# Autodesk Inventor assembly: Durometer_Vertical_Lead_Screw_Assembly
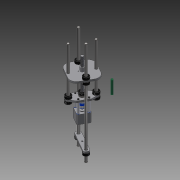
[picture p0: Inventor's stored thumbnail of the model, 180x180]
Saved by Autodesk Inventor 2015 (Build 190159000, 159)
## iProperties
Created: 2014-12-22
Part Number: Durometer_Vertical_Lead_Screw_Assembly
Document SubType Name: Assembly
Designer: Drew
Author: Drew
## Documents named in this file (16)
- C:\Users\Drew\Dropbox\Durometer\Durometer_Assembly\Durometer_Vertical_Lead_Screw_Assembly.iam
- C:\Users\Drew\Dropbox\Durometer\Durometer_Assembly\Stepper_Motor.ipt
- C:\Users\Drew\Dropbox\Durometer\Durometer_Assembly\Shaft_Coupler_5mm_10mm.ipt
- C:\Users\Drew\Dropbox\Durometer\Durometer_Assembly\Lead_Screw_10x2.ipt
- C:\Users\Drew\Dropbox\Durometer\Durometer_Assembly\Thrust_Bearing_6655K550.ipt
- C:\Users\Drew\Dropbox\Durometer\Durometer_Assembly\Shaft_Collar_6063K150.ipt
- C:\Users\Drew\Dropbox\Durometer\Durometer_Assembly\Vertical_Lead_Screw_Shaft_Mount_Plate_Mid.ipt
- C:\Users\Drew\Dropbox\Durometer\Durometer_Assembly\M3_40mm_Spacer_92871A217.ipt
- C:\Users\Drew\Dropbox\Durometer\Durometer_Assembly\M3_Screw_50mm_91290A137.ipt
- C:\Users\Drew\Dropbox\Durometer\Durometer_Assembly\Lead_Screw_Flange_Nut.ipt
- C:\Users\Drew\Dropbox\Durometer\Durometer_Assembly\Shaft_200mm_6112K101.ipt
- C:\Users\Drew\Dropbox\Durometer\Durometer_Assembly\Vertical_Lead_Screw_Plate.ipt
- C:\Users\Drew\Dropbox\Durometer\Durometer_Assembly\Shaft_400mm_6112K102.ipt
- C:\Users\Drew\Dropbox\Durometer\Durometer_Assembly\Shaft_Collar_57485K680.ipt
- C:\Users\Drew\Dropbox\Durometer\Durometer_Assembly\Support_Plate.ipt
- C:\Users\Drew\Dropbox\Durometer\Durometer_Assembly\8-32_Spacer_50mm.ipt
## Components (33 placed, 15 different names)
1. Stepper_Motor:1 — Mate:1, Mate:2, Mate:20, Mate:21, Mate:22, Mate:23, Mate:24, Mate:25, Mate:26, Mate:27, Mate:28
2. Shaft_Coupler_5mm_10mm:1 — Mate:1, Mate:2, Mate:3, Mate:4, Mate:6
3. Lead_Screw_10x2:1 — Mate:3, Mate:4, Mate:5, Mate:7, Mate:12, Mate:37, Mate:40
4. Thrust_Bearing_6655K550:1 — Mate:7, Mate:8, Mate:9, Mate:18
5. Thrust_Bearing_6655K550:2 — Mate:5, Mate:6, Mate:19
6. Shaft_Collar_6063K150:1 — Mate:8, Mate:9
7. Vertical_Lead_Screw_Shaft_Mount_Plate_Mid:1 — Mate:12, Mate:18, Mate:19, Mate:20, Mate:29, Mate:30, Mate:31, Mate:32, Mate:38, Mate:39, Mate:66, Mate:67, Mate:68, Mate:69
8. M3_40mm_Spacer_92871A217:1 — Mate:21, Mate:22, Mate:33
9. M3_40mm_Spacer_92871A217:2 — Mate:23, Mate:24, Mate:36
10. M3_40mm_Spacer_92871A217:3 — Mate:25, Mate:26, Mate:34
11. M3_40mm_Spacer_92871A217:4 — Mate:27, Mate:28, Mate:35
12. M3_Screw_50mm_91290A137:1 — Mate:30, Mate:36
13. M3_Screw_50mm_91290A137:2 — Mate:31, Mate:34
14. M3_Screw_50mm_91290A137:3 — Mate:32, Mate:33
15. M3_Screw_50mm_91290A137:4 — Mate:29, Mate:35
16. Lead_Screw_Flange_Nut:1 — Mate:37, Mate:70, Mate:71
17. Shaft_200mm_6112K101:1 — Mate:38, Mate:41, Mate:64, Mate:65, Flush:1
18. Shaft_200mm_6112K101:2 — Mate:39, Mate:62, Mate:63, Flush:2
19. Vertical_Lead_Screw_Plate:1 — Mate:40, Mate:41, Mate:42, Mate:43, Mate:46, Mate:47, Mate:50, Mate:51, Mate:70, Mate:71
20. Shaft_400mm_6112K102:1 — Mate:43, Mate:45, Mate:48, Mate:53, Mate:56
21. Shaft_400mm_6112K102:2 — Mate:42, Mate:44, Mate:49, Mate:55, Mate:73
22. Shaft_Collar_57485K680:1 — Mate:45, Mate:47
23. Shaft_Collar_57485K680:2 — Mate:44, Mate:46
24. Shaft_Collar_57485K680:3 — Mate:49, Mate:51
25. Shaft_Collar_57485K680:4 — Mate:48, Mate:50
26. Shaft_Collar_57485K680:6 — Mate:55, Mate:60
27. Shaft_Collar_57485K680:7 — Mate:53, Mate:58
28. Support_Plate:1 — Mate:56, Mate:58, Mate:60, Mate:73
29. Shaft_Collar_57485K680:9 — Mate:62, Mate:66, Flush:2
30. Shaft_Collar_57485K680:10 — Mate:63, Mate:67
31. Shaft_Collar_57485K680:11 — Mate:65, Mate:68
32. Shaft_Collar_57485K680:12 — Mate:64, Mate:69, Flush:1
33. 8-32_Spacer_50mm:1
## Relationships (62: Mate 60, Flush 2)
- Mate:1: Stepper_Motor:1 ↔ Shaft_Coupler_5mm_10mm:1
- Mate:2 (6.604 mm): Stepper_Motor:1 ↔ Shaft_Coupler_5mm_10mm:1
- Mate:3: Shaft_Coupler_5mm_10mm:1 ↔ Lead_Screw_10x2:1
- Mate:4: Shaft_Coupler_5mm_10mm:1 ↔ Lead_Screw_10x2:1
- Mate:5: Lead_Screw_10x2:1 ↔ Thrust_Bearing_6655K550:2
- Mate:6: Shaft_Coupler_5mm_10mm:1 ↔ Thrust_Bearing_6655K550:2
- Mate:7: Lead_Screw_10x2:1 ↔ Thrust_Bearing_6655K550:1
- Mate:8: Thrust_Bearing_6655K550:1 ↔ Shaft_Collar_6063K150:1
- Mate:9: Thrust_Bearing_6655K550:1 ↔ Shaft_Collar_6063K150:1
- Mate:12: Lead_Screw_10x2:1 ↔ Vertical_Lead_Screw_Shaft_Mount_Plate_Mid:1
- Mate:18: Thrust_Bearing_6655K550:1 ↔ Vertical_Lead_Screw_Shaft_Mount_Plate_Mid:1
- Mate:19: Thrust_Bearing_6655K550:2 ↔ Vertical_Lead_Screw_Shaft_Mount_Plate_Mid:1
- Mate:20: Stepper_Motor:1 ↔ Vertical_Lead_Screw_Shaft_Mount_Plate_Mid:1
- Mate:21: Stepper_Motor:1 ↔ M3_40mm_Spacer_92871A217:1
- Mate:22: Stepper_Motor:1 ↔ M3_40mm_Spacer_92871A217:1
- Mate:23: Stepper_Motor:1 ↔ M3_40mm_Spacer_92871A217:2
- Mate:24: Stepper_Motor:1 ↔ M3_40mm_Spacer_92871A217:2
- Mate:25: Stepper_Motor:1 ↔ M3_40mm_Spacer_92871A217:3
- Mate:26: Stepper_Motor:1 ↔ M3_40mm_Spacer_92871A217:3
- Mate:27: Stepper_Motor:1 ↔ M3_40mm_Spacer_92871A217:4
- Mate:28: Stepper_Motor:1 ↔ M3_40mm_Spacer_92871A217:4
- Mate:29: Vertical_Lead_Screw_Shaft_Mount_Plate_Mid:1 ↔ M3_Screw_50mm_91290A137:4
- Mate:30: Vertical_Lead_Screw_Shaft_Mount_Plate_Mid:1 ↔ M3_Screw_50mm_91290A137:1
- Mate:31: Vertical_Lead_Screw_Shaft_Mount_Plate_Mid:1 ↔ M3_Screw_50mm_91290A137:2
- Mate:32: Vertical_Lead_Screw_Shaft_Mount_Plate_Mid:1 ↔ M3_Screw_50mm_91290A137:3
- Mate:33: M3_40mm_Spacer_92871A217:1 ↔ M3_Screw_50mm_91290A137:3
- Mate:34: M3_40mm_Spacer_92871A217:3 ↔ M3_Screw_50mm_91290A137:2
- Mate:35: M3_40mm_Spacer_92871A217:4 ↔ M3_Screw_50mm_91290A137:4
- Mate:36: M3_40mm_Spacer_92871A217:2 ↔ M3_Screw_50mm_91290A137:1
- Mate:37: Lead_Screw_10x2:1 ↔ Lead_Screw_Flange_Nut:1
- Mate:38: Vertical_Lead_Screw_Shaft_Mount_Plate_Mid:1 ↔ Shaft_200mm_6112K101:1
- Mate:39: Vertical_Lead_Screw_Shaft_Mount_Plate_Mid:1 ↔ Shaft_200mm_6112K101:2
- Mate:40: Lead_Screw_10x2:1 ↔ Vertical_Lead_Screw_Plate:1
- Mate:41: Shaft_200mm_6112K101:1 ↔ Vertical_Lead_Screw_Plate:1
- Mate:42: Vertical_Lead_Screw_Plate:1 ↔ Shaft_400mm_6112K102:2
- Mate:43: Vertical_Lead_Screw_Plate:1 ↔ Shaft_400mm_6112K102:1
- Mate:44: Shaft_400mm_6112K102:2 ↔ Shaft_Collar_57485K680:2
- Mate:45: Shaft_400mm_6112K102:1 ↔ Shaft_Collar_57485K680:1
- Mate:46: Vertical_Lead_Screw_Plate:1 ↔ Shaft_Collar_57485K680:2
- Mate:47: Vertical_Lead_Screw_Plate:1 ↔ Shaft_Collar_57485K680:1
- Mate:48: Shaft_400mm_6112K102:1 ↔ Shaft_Collar_57485K680:4
- Mate:49: Shaft_400mm_6112K102:2 ↔ Shaft_Collar_57485K680:3
- Mate:50: Vertical_Lead_Screw_Plate:1 ↔ Shaft_Collar_57485K680:4
- Mate:51: Vertical_Lead_Screw_Plate:1 ↔ Shaft_Collar_57485K680:3
- Mate:53: Shaft_400mm_6112K102:1 ↔ Shaft_Collar_57485K680:7
- Mate:55: Shaft_400mm_6112K102:2 ↔ Shaft_Collar_57485K680:6
- Mate:56: Shaft_400mm_6112K102:1 ↔ Support_Plate:1
- Mate:58: Shaft_Collar_57485K680:7 ↔ Support_Plate:1
- Mate:60: Shaft_Collar_57485K680:6 ↔ Support_Plate:1
- Mate:62: Shaft_200mm_6112K101:2 ↔ Shaft_Collar_57485K680:9
- Mate:63: Shaft_200mm_6112K101:2 ↔ Shaft_Collar_57485K680:10
- Mate:64: Shaft_200mm_6112K101:1 ↔ Shaft_Collar_57485K680:12
- Mate:65: Shaft_200mm_6112K101:1 ↔ Shaft_Collar_57485K680:11
- Mate:66: Vertical_Lead_Screw_Shaft_Mount_Plate_Mid:1 ↔ Shaft_Collar_57485K680:9
- Mate:67: Vertical_Lead_Screw_Shaft_Mount_Plate_Mid:1 ↔ Shaft_Collar_57485K680:10
- Mate:68: Vertical_Lead_Screw_Shaft_Mount_Plate_Mid:1 ↔ Shaft_Collar_57485K680:11
- Mate:69: Vertical_Lead_Screw_Shaft_Mount_Plate_Mid:1 ↔ Shaft_Collar_57485K680:12
- Mate:70: Lead_Screw_Flange_Nut:1 ↔ Vertical_Lead_Screw_Plate:1
- Mate:71: Lead_Screw_Flange_Nut:1 ↔ Vertical_Lead_Screw_Plate:1
- Mate:73: Shaft_400mm_6112K102:2 ↔ Support_Plate:1
- Flush:1: Shaft_200mm_6112K101:1 ↔ Shaft_Collar_57485K680:12
- Flush:2: Shaft_200mm_6112K101:2 ↔ Shaft_Collar_57485K680:9
